# Autodesk Inventor assembly: Perfect Square Compartment Frame
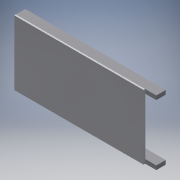
[picture p0: Inventor's stored thumbnail of the model, 180x180]
Saved by Autodesk Inventor 2017 (Build 210142000, 142)
## iProperties
Created: 2017-05-30
Part Number: Perfect Square Compartment Frame
Document SubType Name: Assembly
Designer: cas7
Author: cas7
## Documents named in this file (3)
- C:\Users\Public\Documents\Autodesk\.desktop-connect\.docstore\guided-tutorial-plugin\INVNTOR\Compartment Modeling\Perfect Square Compartment Frame.iam
- C:\Users\Public\Documents\Autodesk\.desktop-connect\.docstore\guided-tutorial-plugin\INVNTOR\Compartment Modeling\52.125 2x4.ipt
- C:\Users\Public\Documents\Autodesk\.desktop-connect\.docstore\guided-tutorial-plugin\INVNTOR\2017\ENU\552100320579484105\TutorialModelPath\4x2 Gyp Board.ipt
## Components (3 placed, 2 different names)
1. 52.125 2x4:1 — Mate:1, Mate:2, Mate:3
2. 52.125 2x4:2 — Mate:4, Mate:5
3. 4x2 Gyp Board:1 — Mate:1, Mate:2, Mate:3, Mate:4, Mate:5
## Relationships (5: Mate 5)
- Mate:1: 52.125 2x4:1 ↔ 4x2 Gyp Board:1
- Mate:2: 52.125 2x4:1 ↔ 4x2 Gyp Board:1
- Mate:3: 52.125 2x4:1 ↔ 4x2 Gyp Board:1
- Mate:4: 52.125 2x4:2 ↔ 4x2 Gyp Board:1
- Mate:5: 52.125 2x4:2 ↔ 4x2 Gyp Board:1
